# Autodesk Inventor assembly: Hotend Assembly
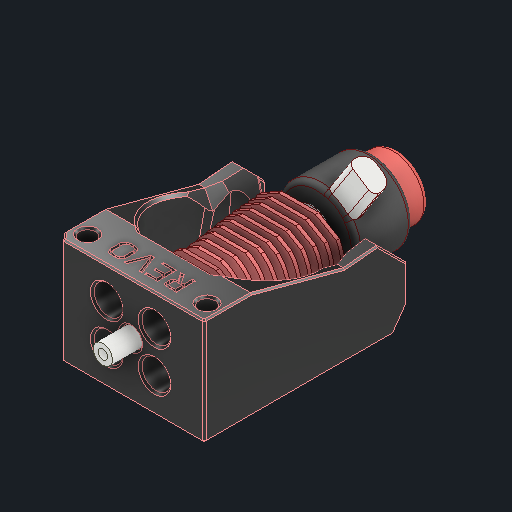
[picture p0: Inventor's stored thumbnail of the model, 512x512]
Saved by Autodesk Inventor 2025.1 (Build 291241020, 241B)
## iProperties
Created: 2025-05-09
Part Number: Hotend Assembly
Document SubType Name: Assembly
Designer: AdminForWorker
Title: Hotend Assembly
Author: AdminForWorker
## Documents named in this file (5)
- C:\Users\Joshua Eah\Documents\Voron 0.2\CAD\Master Assembly\Toolhead\Hotend Assembly.iam
- C:\Users\Joshua Eah\Documents\Voron 0.2\CAD\Master Assembly\PTFE Tube.ipt
- C:\Users\Joshua Eah\Documents\Voron 0.2\CAD\Master Assembly\Revo Voron Mount.ipt
- C:\Users\Joshua Eah\Documents\Voron 0.2\CAD\Master Assembly\Toolhead\Hotend.ipt
- C:\Users\Joshua Eah\Documents\Voron 0.2\CAD\Master Assembly\Hardware\M3x8 BHCS.ipt
## Components (7 placed, 4 different names)
1. PTFE Tube:1 — Insert:1
2. Revo Voron Mount:1 — Insert:2, Insert:3, Insert:4, Insert:5
3. Hotend — Insert:1
4. M3x8 BHCS:1 — Insert:2
5. M3x8 BHCS:2 — Insert:3
6. M3x8 BHCS:3 — Insert:5
7. M3x8 BHCS:4 — Insert:4
## Relationships (5: Insert 5)
- Insert:1: PTFE Tube:1 ↔ Hotend
- Insert:2: Revo Voron Mount:1 ↔ M3x8 BHCS:1
- Insert:3: Revo Voron Mount:1 ↔ M3x8 BHCS:2
- Insert:4: Revo Voron Mount:1 ↔ M3x8 BHCS:4
- Insert:5: Revo Voron Mount:1 ↔ M3x8 BHCS:3
